# Autodesk Inventor assembly: HopperAssembly42inch_v5
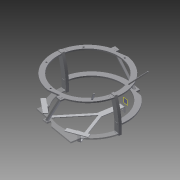
[picture p0: Inventor's stored thumbnail of the model, 180x180]
Saved by Autodesk Inventor 2013 (Build 170138000, 138)
## iProperties
Created: 2013-01-17
Part Number: HopperAssembly42inch_v5
Document SubType Name: Assembly
Designer: twsass
Mass: 535.116 g
Surface Area: 1960.7 cm^2
Volume: 456.721 cm^3
Density: 1.17165 g/cm^3
Author: twsass
## Documents named in this file (9)
- \\NNHSSRV2.hs.sd203.org\ACToennies$\Robotics\Hopper\HopperAssembly42inch_v5.iam
- \\NNHSSRV2.hs.sd203.org\ACToennies$\Robotics\Hopper\TopHoopSection_v4.ipt
- \\NNHSSRV2.hs.sd203.org\ACToennies$\Robotics\Hopper\HopperFrontSupport_v2.ipt
- \\NNHSSRV2.hs.sd203.org\ACToennies$\Robotics\Hopper\BottomHoop_v1.ipt
- \\NNHSSRV2.hs.sd203.org\ACToennies$\Robotics\Hopper\MiddleHoop.ipt
- \\NNHSSRV2.hs.sd203.org\ACToennies$\Robotics\Hopper\1Piecelongsupport_v1.ipt
- \\NNHSSRV2.hs.sd203.org\ACToennies$\Robotics\Hopper\1Pieceshortsupport_v1.ipt
- \\NNHSSRV2.hs.sd203.org\ACToennies$\Robotics\Hopper\Funneling_v1.ipt
- \\NNHSSRV2.hs.sd203.org\ACToennies$\Robotics\Hopper\Feeder-Grabber_v2.ipt
## Components (11 placed, 8 different names)
1. TopHoopSection_v4:1 — Mate:113, Mate:114, Mate:115, Flush:1, Mate:122, Mate:123, Mate:140, Mate:141, Flush:3, Mate:143, Mate:144
2. HopperFrontSupport_v2:2 — Mate:116, Mate:117, Mate:118, Mate:122, Mate:128, Mate:129, Mate:130, Flush:2
3. TopHoopSection_v4:2 — Mate:116, Mate:117, Mate:118, Flush:1, Mate:123, Mate:124, Mate:125, Mate:126, Mate:145, Mate:146, Flush:4
4. MiddleHoop:1 — Mate:119, Mate:120, Mate:121
5. HopperFrontSupport_v2:3 — Mate:113, Mate:114, Mate:115, Mate:119, Mate:120, Mate:121, Mate:127
6. 1Pieceshortsupport_v1:1 — Mate:124, Mate:125, Mate:126
7. BottomHoop_v1:1 — Mate:127, Mate:128, Mate:129, Mate:130, Mate:131, Mate:142
8. 1Piecelongsupport_v1:1 — Mate:131, Mate:140, Mate:141
9. Funneling_v1:1 — Mate:145, Mate:146, Flush:4
10. Funneling_v1:2 — Flush:3, Mate:143, Mate:144
11. Feeder-Grabber_v2:1 — Mate:142, Flush:2
## Relationships (30: Mate 26, Flush 4)
- Mate:113: TopHoopSection_v4:1 ↔ HopperFrontSupport_v2:3
- Mate:114: TopHoopSection_v4:1 ↔ HopperFrontSupport_v2:3
- Mate:115: TopHoopSection_v4:1 ↔ HopperFrontSupport_v2:3
- Mate:116: HopperFrontSupport_v2:2 ↔ TopHoopSection_v4:2
- Mate:117: HopperFrontSupport_v2:2 ↔ TopHoopSection_v4:2
- Mate:118: HopperFrontSupport_v2:2 ↔ TopHoopSection_v4:2
- Mate:119: MiddleHoop:1 ↔ HopperFrontSupport_v2:3
- Mate:120: MiddleHoop:1 ↔ HopperFrontSupport_v2:3
- Mate:121: MiddleHoop:1 ↔ HopperFrontSupport_v2:3
- Flush:1: TopHoopSection_v4:1 ↔ TopHoopSection_v4:2
- Mate:122: TopHoopSection_v4:1 ↔ HopperFrontSupport_v2:2
- Mate:123: TopHoopSection_v4:1 ↔ TopHoopSection_v4:2
- Mate:124: TopHoopSection_v4:2 ↔ 1Pieceshortsupport_v1:1
- Mate:125: TopHoopSection_v4:2 ↔ 1Pieceshortsupport_v1:1
- Mate:126: TopHoopSection_v4:2 ↔ 1Pieceshortsupport_v1:1
- Mate:127: HopperFrontSupport_v2:3 ↔ BottomHoop_v1:1
- Mate:128: HopperFrontSupport_v2:2 ↔ BottomHoop_v1:1
- Mate:129: HopperFrontSupport_v2:2 ↔ BottomHoop_v1:1
- Mate:130: HopperFrontSupport_v2:2 ↔ BottomHoop_v1:1
- Mate:131: BottomHoop_v1:1 ↔ 1Piecelongsupport_v1:1
- Mate:140: TopHoopSection_v4:1 ↔ 1Piecelongsupport_v1:1
- Mate:141: TopHoopSection_v4:1 ↔ 1Piecelongsupport_v1:1
- Mate:142 (-41.275 mm): BottomHoop_v1:1 ↔ Feeder-Grabber_v2:1
- Flush:2 (157.48 mm): HopperFrontSupport_v2:2 ↔ Feeder-Grabber_v2:1
- Flush:3: TopHoopSection_v4:1 ↔ Funneling_v1:2
- Mate:143: TopHoopSection_v4:1 ↔ Funneling_v1:2
- Mate:144: TopHoopSection_v4:1 ↔ Funneling_v1:2
- Mate:145: TopHoopSection_v4:2 ↔ Funneling_v1:1
- Mate:146: TopHoopSection_v4:2 ↔ Funneling_v1:1
- Flush:4: TopHoopSection_v4:2 ↔ Funneling_v1:1
